# Autodesk Inventor assembly: 90-Degree-Metal-Corner
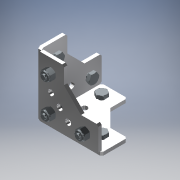
[picture p0: Inventor's stored thumbnail of the model, 180x180]
Saved by Autodesk Inventor 2017.3 (Build 213256000, 256)
## iProperties
Created: 2018-01-04
Part Number: 90-Degree-Metal-Corner
Document SubType Name: Assembly
Designer: pranav
Author: pranav
## iProperties of the stored document REV-41-1361 Simple.ipt
Created: 2017-04-10
Part Number: REV-41-1361 Simple
Material: Generic
Document SubType Name: Modeling
Designer: pranav
Density: 1 g/cm^3
Appearance: Default
Sending System: Autodesk Translation Framework v5.2.0.2920
Preprocessor: ST-DEVELOPER v16.5
Title: E:/Dropbox/REV Robotics/STEP Files/REV-41-1361 Simple.step
## iProperties of the stored document REV-41-1019.ipt
Created: 2015-08-20
Part Number: REV-41-1019
Material: Generic
Description: STEP AP214
Document SubType Name: Modeling
Designer: pranav
Density: 1 g/cm^3
Appearance: Default
Sending System: SolidWorks 2014
Preprocessor: SwSTEP 2.0
Title: REV-41-1019_10mm.STEP
Revision Number: ANY
## iProperties of the stored document REV-41-1359 Simple.ipt
Created: 2017-04-10
Part Number: REV-41-1359 Simple
Material: Generic
Document SubType Name: Modeling
Designer: pranav
Density: 1 g/cm^3
Appearance: Default
Sending System: Autodesk Translation Framework v5.2.0.2920
Preprocessor: ST-DEVELOPER v16.5
Title: E:/Dropbox/REV Robotics/STEP Files/REV-41-1359 Simple.step
## Documents named in this file (8)
- **C:\Users\pranav\Documents\Inventor\REV-Robot-CAD\3D-Metal-Corner.iam*LocalDocs*xOi4pobldP3yuungbIvsvnjgzNd*REV-41-1361 Simple.ipt
- **C:\Users\pranav\Documents\Inventor\REV-Robot-CAD\90-Degree-Metal-Corner.iam*LocalDocs*xEwiivjkf3oheuscs3k0ygyekJg*REV-41-1019.ipt
- **C:\Users\pranav\Documents\Inventor\REV-Robot-CAD\3D-Metal-Corner.iam*LocalDocs*xOsm31qbt01kgeigc3lhdl1n2Ie*REV-41-1359 Simple.ipt
- C:\Users\pranav\Documents\Inventor\REV-Robot-CAD\3D-Metal-Corner.iam
- **C:\Users\pranav\Documents\Inventor\REV-Robot-CAD\3D-Metal-Corner.iam*LocalDocs*xEwiivjkf3oheuscs3k0ygyekJg*REV-41-1019.ipt
- C:\Users\pranav\Documents\Inventor\REV-Robot-CAD\REV Robotics\REV Robotics CAD\REV-41-1019.STEP
- C:\Users\pranav\Documents\Inventor\REV-Robot-CAD\REV Robotics\REV Robotics CAD\REV-41-1359 Simple.step
- C:\Users\pranav\Documents\Inventor\REV-Robot-CAD\REV Robotics\REV Robotics CAD\REV-41-1361 Simple.step
## Components (21 placed, 3 different names)
1. REV-41-1019:1 — Mate:10, Mate:12, Mate:14, Mate:39, Mate:41, Mate:43
2. REV-41-1019:2 — Mate:22, Mate:24, Mate:26, Mate:27, Mate:29, Mate:31
3. REV-41-1019:3 — Mate:16, Mate:18, Mate:20, Mate:33, Mate:35, Mate:37
4. REV-41-1359 Simple:1 — Mate:18, Mate:36
5. REV-41-1359 Simple:2 — Mate:24, Mate:32
6. REV-41-1359 Simple:3 — Mate:10, Mate:40
7. REV-41-1359 Simple:4 — Mate:20, Mate:34
8. REV-41-1359 Simple:5 — Mate:26, Mate:28
9. REV-41-1359 Simple:6 — Mate:22, Mate:30
10. REV-41-1359 Simple:7 — Mate:12, Mate:44
11. REV-41-1359 Simple:8 — Mate:16, Mate:38
12. REV-41-1359 Simple:9 — Mate:14, Mate:42
13. REV-41-1361 Simple:1 — Mate:43, Mate:44
14. REV-41-1361 Simple:2 — Mate:41, Mate:42
15. REV-41-1361 Simple:3 — Mate:37, Mate:38
16. REV-41-1361 Simple:4 — Mate:39, Mate:40
17. REV-41-1361 Simple:5 — Mate:35, Mate:36
18. REV-41-1361 Simple:6 — Mate:33, Mate:34
19. REV-41-1361 Simple:7 — Mate:27, Mate:28
20. REV-41-1361 Simple:8 — Mate:29, Mate:30
21. REV-41-1361 Simple:9 — Mate:31, Mate:32
## Relationships (27: Mate 27)
- Mate:10: REV-41-1019:1 ↔ REV-41-1359 Simple:3
- Mate:12: REV-41-1019:1 ↔ REV-41-1359 Simple:7
- Mate:14: REV-41-1019:1 ↔ REV-41-1359 Simple:9
- Mate:16: REV-41-1019:3 ↔ REV-41-1359 Simple:8
- Mate:18: REV-41-1019:3 ↔ REV-41-1359 Simple:1
- Mate:20: REV-41-1019:3 ↔ REV-41-1359 Simple:4
- Mate:22: REV-41-1019:2 ↔ REV-41-1359 Simple:6
- Mate:24: REV-41-1019:2 ↔ REV-41-1359 Simple:2
- Mate:26: REV-41-1019:2 ↔ REV-41-1359 Simple:5
- Mate:27: REV-41-1019:2 ↔ REV-41-1361 Simple:7
- Mate:28: REV-41-1359 Simple:5 ↔ REV-41-1361 Simple:7
- Mate:29: REV-41-1019:2 ↔ REV-41-1361 Simple:8
- Mate:30: REV-41-1359 Simple:6 ↔ REV-41-1361 Simple:8
- Mate:31: REV-41-1019:2 ↔ REV-41-1361 Simple:9
- Mate:32: REV-41-1359 Simple:2 ↔ REV-41-1361 Simple:9
- Mate:33: REV-41-1019:3 ↔ REV-41-1361 Simple:6
- Mate:34: REV-41-1359 Simple:4 ↔ REV-41-1361 Simple:6
- Mate:35: REV-41-1019:3 ↔ REV-41-1361 Simple:5
- Mate:36: REV-41-1359 Simple:1 ↔ REV-41-1361 Simple:5
- Mate:37: REV-41-1019:3 ↔ REV-41-1361 Simple:3
- Mate:38: REV-41-1359 Simple:8 ↔ REV-41-1361 Simple:3
- Mate:39: REV-41-1019:1 ↔ REV-41-1361 Simple:4
- Mate:40: REV-41-1359 Simple:3 ↔ REV-41-1361 Simple:4
- Mate:41: REV-41-1019:1 ↔ REV-41-1361 Simple:2
- Mate:42: REV-41-1359 Simple:9 ↔ REV-41-1361 Simple:2
- Mate:43: REV-41-1019:1 ↔ REV-41-1361 Simple:1
- Mate:44: REV-41-1359 Simple:7 ↔ REV-41-1361 Simple:1
